# Autodesk Inventor assembly: Baldachin
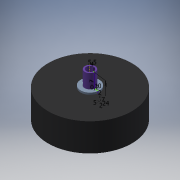
[picture p0: Inventor's stored thumbnail of the model, 180x180]
Saved by Autodesk Inventor 2018.2 (Build 222227000, 227)
## iProperties
Created: 2018-03-05
Part Number: Baldachin
Material: Generisch
Document SubType Name: Assembly
Designer: JochenAlt
Author: JochenAlt
## Documents named in this file (3)
- D:\Projects\concretelamp\CAD\Baldachin.iam
- D:\Projects\Donna\CAD\Baldachin Form.ipt
- D:\Projects\concretelamp\CAD\Zugentlastung.ipt
## Components (2 placed, 2 different names)
1. Baldachin Form:1 — Passend:1, Passend:2
2. Zugentlastung:1 — Passend:1, Passend:2
## Relationships (2: Mate 2)
- Passend:1 [Mate]: Baldachin Form:1 ↔ Zugentlastung:1
- Passend:2 [Mate]: Baldachin Form:1 ↔ Zugentlastung:1
